# Autodesk Inventor assembly: ч ASY human dummy 01
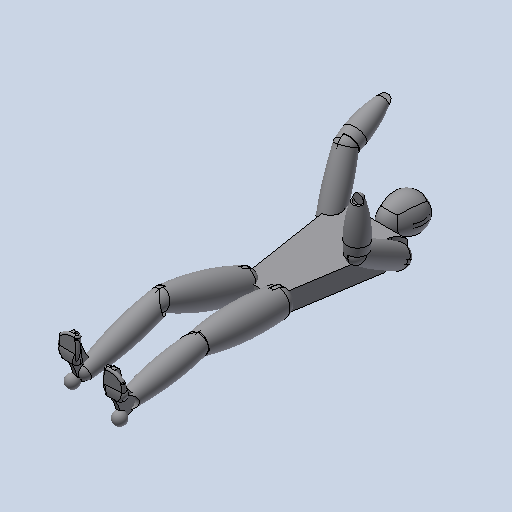
[picture p0: Inventor's stored thumbnail of the model, 512x512]
Saved by Autodesk Inventor 2025.1 (Build 291241020, 241B)
## iProperties
Created: 2018-05-21
Part Number: ч ASY human dummy 01
Material: Типовые
Document SubType Name: Assembly
Designer: admin
Stock Number: ч ASY human dummy 01
Description: Dummy
Author: admin
Revision Number: 1
## Documents named in this file (12)
- C:\Users\user\YandexDisk-badmisterfox\домашниий пк\Inventor\NDM-VOS_powder_hopper\human 01\ч ASY human dummy 01.iam
- C:\Users\user\YandexDisk-badmisterfox\домашниий пк\Inventor\NDM-VOS_powder_hopper\human 01\shoulder joint.ipt
- C:\Users\user\YandexDisk-badmisterfox\домашниий пк\Inventor\NDM-VOS_powder_hopper\human 01\Shoulder parametric.ipt
- C:\Users\user\YandexDisk-badmisterfox\домашниий пк\Inventor\NDM-VOS_powder_hopper\human 01\body parametric.ipt
- C:\Users\user\YandexDisk-badmisterfox\домашниий пк\Inventor\NDM-VOS_powder_hopper\human 01\feet parametric.ipt
- C:\Users\user\YandexDisk-badmisterfox\домашниий пк\Inventor\NDM-VOS_powder_hopper\human 01\Forearm.ipt
- C:\Users\user\YandexDisk-badmisterfox\домашниий пк\Inventor\NDM-VOS_powder_hopper\human 01\Elbow.ipt
- C:\Users\user\YandexDisk-badmisterfox\домашниий пк\Inventor\NDM-VOS_powder_hopper\human 01\Hip.ipt
- C:\Users\user\YandexDisk-badmisterfox\домашниий пк\Inventor\NDM-VOS_powder_hopper\human 01\upper leg.ipt
- C:\Users\user\YandexDisk-badmisterfox\домашниий пк\Inventor\NDM-VOS_powder_hopper\human 01\shank.ipt
- C:\Users\user\YandexDisk-badmisterfox\домашниий пк\Inventor\NDM-VOS_powder_hopper\human 01\feet parametric_MIR.ipt
- C:\Users\user\YandexDisk-badmisterfox\домашниий пк\Inventor\NDM-VOS_powder_hopper\human 01\Head.ipt
## Components (18 placed, 11 different names)
1. shoulder joint.ipt:1 — С поворотом:1, С поворотом:9
2. Shoulder parametric.ipt:1 — С поворотом:1, С поворотом:3
3. body parametric.ipt:1 — Заподлицо:2, С поворотом:9, Заподлицо:7, Заподлицо:8, С поворотом:10, С поворотом:14, С поворотом:15, Совмещение:1, Заподлицо:10
4. feet parametric.ipt:1 — С поворотом:20
5. Forearm.ipt:1 — С поворотом:2
6. Elbow.ipt:1 — С поворотом:2, С поворотом:3
7. Hip.ipt:1 — С поворотом:14, С поворотом:19
8. upper leg.ipt:1 — С поворотом:19, С поворотом:17
9. upper leg.ipt:2 — С поворотом:18, С поворотом:16
10. Hip.ipt:2 — С поворотом:15, С поворотом:18
11. shank.ipt:1 — С поворотом:16, С поворотом:20
12. shank.ipt:2 — С поворотом:17, С поворотом:21
13. shoulder joint.ipt:2 — С поворотом:10, С поворотом:11
14. Shoulder parametric.ipt:2 — С поворотом:11, С поворотом:13
15. Elbow.ipt:2 — С поворотом:12, С поворотом:13
16. Forearm.ipt:2 — С поворотом:12
17. feet parametric_MIR.ipt:1 — С поворотом:21
18. Head.ipt:1 — Заподлицо:9, Совмещение:1, Заподлицо:10
## Relationships (22: RevoluteJoint 16, Flush 5, Mate 1)
- С поворотом:1 [RevoluteJoint]: shoulder joint.ipt:1 ↔ Shoulder parametric.ipt:1
- Заподлицо:2 [Flush]: body parametric.ipt:1
- С поворотом:2 [RevoluteJoint]: Forearm.ipt:1 ↔ Elbow.ipt:1
- С поворотом:3 [RevoluteJoint]: Shoulder parametric.ipt:1 ↔ Elbow.ipt:1
- С поворотом:9 [RevoluteJoint]: shoulder joint.ipt:1 ↔ body parametric.ipt:1
- Заподлицо:7 [Flush]: body parametric.ipt:1
- Заподлицо:8 [Flush]: body parametric.ipt:1
- С поворотом:10 [RevoluteJoint]: body parametric.ipt:1 ↔ shoulder joint.ipt:2
- С поворотом:11 [RevoluteJoint]: shoulder joint.ipt:2 ↔ Shoulder parametric.ipt:2
- С поворотом:12 [RevoluteJoint]: Elbow.ipt:2 ↔ Forearm.ipt:2
- С поворотом:13 [RevoluteJoint]: Shoulder parametric.ipt:2 ↔ Elbow.ipt:2
- С поворотом:14 [RevoluteJoint]: body parametric.ipt:1 ↔ Hip.ipt:1
- С поворотом:15 [RevoluteJoint]: body parametric.ipt:1 ↔ Hip.ipt:2
- С поворотом:19 [RevoluteJoint]: Hip.ipt:1 ↔ upper leg.ipt:1
- С поворотом:18 [RevoluteJoint]: upper leg.ipt:2 ↔ Hip.ipt:2
- С поворотом:16 [RevoluteJoint]: upper leg.ipt:2 ↔ shank.ipt:1
- С поворотом:17 [RevoluteJoint]: upper leg.ipt:1 ↔ shank.ipt:2
- С поворотом:20 [RevoluteJoint]: feet parametric.ipt:1 ↔ shank.ipt:1
- С поворотом:21 [RevoluteJoint]: shank.ipt:2 ↔ feet parametric_MIR.ipt:1
- Заподлицо:9 [Flush]: Head.ipt:1
- Совмещение:1 [Mate] (100 mm): body parametric.ipt:1 ↔ Head.ipt:1
- Заподлицо:10 [Flush]: body parametric.ipt:1 ↔ Head.ipt:1
